# Autodesk Inventor assembly: 1x4 Male Header 90'
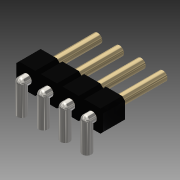
[picture p0: Inventor's stored thumbnail of the model, 180x180]
Saved by Autodesk Inventor 2015 (Build 190159000, 159)
## iProperties
Created: 2016-01-20
Part Number: 1x4 Male Header 90'
Document SubType Name: Assembly
Designer: Kyle
Author: Kyle
## Documents named in this file (2)
- C:\Users\Kyle\Documents\Autodesk\Output\Inventor 2015\Electronics\Headers\Male\1x4 Male Header 90'.iam
- C:\Users\Kyle\Documents\Autodesk\Output\Inventor 2015\Electronics\Headers\Male\1x1 Male Header 90'.iam
## Components (4 placed, 1 different names)
1. 1x1 Male Header 90':1 [sub-assembly] — Mate:1, Mate:2, Flush:1, Flush:2, Flush:4, Flush:5
2. 1x1 Male Header 90':2 [sub-assembly] — Mate:1, Flush:1, Flush:4
3. 1x1 Male Header 90':3 [sub-assembly] — Mate:2, Mate:3, Flush:2, Flush:3, Flush:5, Flush:6
4. 1x1 Male Header 90':4 [sub-assembly] — Mate:3, Flush:3, Flush:6
## Relationships (9: Flush 6, Mate 3)
- Mate:1: 1x1 Male Header 90':1 ↔ 1x1 Male Header 90':2
- Mate:2: 1x1 Male Header 90':1 ↔ 1x1 Male Header 90':3
- Mate:3: 1x1 Male Header 90':3 ↔ 1x1 Male Header 90':4
- Flush:1: 1x1 Male Header 90':1 ↔ 1x1 Male Header 90':2
- Flush:2: 1x1 Male Header 90':1 ↔ 1x1 Male Header 90':3
- Flush:3: 1x1 Male Header 90':3 ↔ 1x1 Male Header 90':4
- Flush:4: 1x1 Male Header 90':1 ↔ 1x1 Male Header 90':2
- Flush:5: 1x1 Male Header 90':1 ↔ 1x1 Male Header 90':3
- Flush:6: 1x1 Male Header 90':3 ↔ 1x1 Male Header 90':4
